# Autodesk Inventor assembly: nc_nhk8
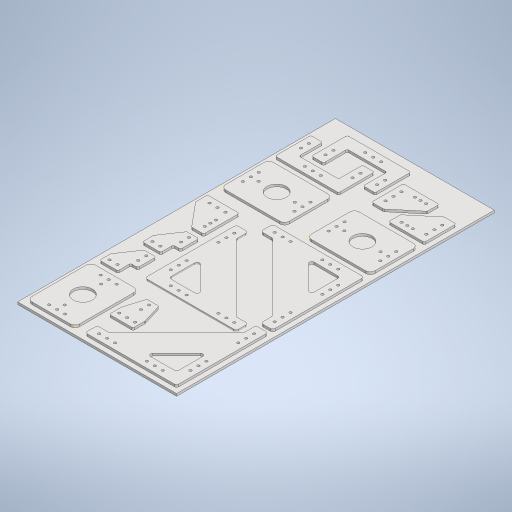
[picture p0: Inventor's stored thumbnail of the model, 512x512]
Saved by Autodesk Inventor 2023 (Build 270158000, 158)
## iProperties
Created: 2022-04-21
Part Number: nc_nhk8
Document SubType Name: Assembly
Designer: yuta
Author: yuta
## Documents named in this file (8)
- C:\Users\yuta\Documents\NHK\nc_nhk8.iam
- C:\Users\yuta\Documents\NHK\NC.port.ipt
- C:\Users\yuta\Documents\NHK\射出_エンコーダー固定.ipt
- C:\Users\yuta\Documents\NHK\射出_固定5.ipt
- C:\Users\yuta\Documents\NHK\射出_固定4.ipt
- C:\Users\yuta\Documents\NHK\射出_固定2.ipt
- C:\Users\yuta\Documents\NHK\射出_固定3.ipt
- C:\Users\yuta\Documents\NHK\射出_固定1.ipt
## Components (15 placed, 7 different names)
1. NC.port:1 — メイト:1, フラッシュ:1, フラッシュ:2, メイト:2, フラッシュ:3, フラッシュ:4, メイト:5, メイト:8, フラッシュ:5, メイト:12, メイト:14, メイト:17, フラッシュ:6, メイト:19, フラッシュ:7, メイト:21, フラッシュ:8, メイト:23, フラッシュ:9, メイト:25, メイト:28, メイト:30, フラッシュ:10
2. 射出_固定5:1 — メイト:5, メイト:6, メイト:7, メイト:10
3. 射出_固定2:1 — メイト:2, フラッシュ:3, フラッシュ:4, メイト:7, メイト:9, メイト:11
4. 射出_エンコーダー固定:1 — メイト:1, フラッシュ:1, フラッシュ:2, メイト:6, メイト:13
5. 射出_固定2:2 — メイト:8, フラッシュ:5, メイト:9, メイト:18, メイト:20
6. 射出_固定2:3 — メイト:10, メイト:11, メイト:16
7. 射出_固定4:1 — メイト:14, メイト:15, メイト:16, メイト:22
8. 射出_固定4:2 — メイト:12, メイト:13, メイト:15
9. 射出_エンコーダー固定:2 — メイト:17, フラッシュ:6, メイト:18, メイト:24
10. 射出_エンコーダー固定:3 — メイト:19, フラッシュ:7, メイト:20, メイト:31
11. 射出_固定3:1 — メイト:21, フラッシュ:8, メイト:22
12. 射出_固定3:2 — メイト:30, フラッシュ:10, メイト:31
13. 射出_固定3:3 — メイト:28, メイト:29
14. 射出_固定1:1 — メイト:25, メイト:26, メイト:27, メイト:29
15. 射出_固定1:2 — メイト:23, メイト:24, フラッシュ:9, メイト:26, メイト:27
## Relationships (39: Mate 29, Flush 10)
- メイト:1 [Mate]: NC.port:1 ↔ 射出_エンコーダー固定:1
- フラッシュ:1 [Flush] (6 mm): NC.port:1 ↔ 射出_エンコーダー固定:1
- フラッシュ:2 [Flush] (6 mm): NC.port:1 ↔ 射出_エンコーダー固定:1
- メイト:2 [Mate]: NC.port:1 ↔ 射出_固定2:1
- フラッシュ:3 [Flush] (6 mm): NC.port:1 ↔ 射出_固定2:1
- フラッシュ:4 [Flush] (6 mm): NC.port:1 ↔ 射出_固定2:1
- メイト:5 [Mate]: NC.port:1 ↔ 射出_固定5:1
- メイト:6 [Mate] (8 mm): 射出_固定5:1 ↔ 射出_エンコーダー固定:1
- メイト:7 [Mate] (10 mm): 射出_固定5:1 ↔ 射出_固定2:1
- メイト:8 [Mate]: NC.port:1 ↔ 射出_固定2:2
- フラッシュ:5 [Flush] (6 mm): NC.port:1 ↔ 射出_固定2:2
- メイト:9 [Mate] (6 mm): 射出_固定2:1 ↔ 射出_固定2:2
- メイト:10 [Mate] (23 mm): 射出_固定5:1 ↔ 射出_固定2:3
- メイト:11 [Mate] (8 mm): 射出_固定2:1 ↔ 射出_固定2:3
- メイト:12 [Mate]: NC.port:1 ↔ 射出_固定4:2
- メイト:13 [Mate] (8 mm): 射出_エンコーダー固定:1 ↔ 射出_固定4:2
- メイト:14 [Mate]: NC.port:1 ↔ 射出_固定4:1
- メイト:15 [Mate] (8 mm): 射出_固定4:1 ↔ 射出_固定4:2
- メイト:16 [Mate] (8 mm): 射出_固定2:3 ↔ 射出_固定4:1
- メイト:17 [Mate]: NC.port:1 ↔ 射出_エンコーダー固定:2
- フラッシュ:6 [Flush] (6 mm): NC.port:1 ↔ 射出_エンコーダー固定:2
- メイト:18 [Mate] (8 mm): 射出_固定2:2 ↔ 射出_エンコーダー固定:2
- メイト:19 [Mate]: NC.port:1 ↔ 射出_エンコーダー固定:3
- フラッシュ:7 [Flush] (6 mm): NC.port:1 ↔ 射出_エンコーダー固定:3
- メイト:20 [Mate] (8 mm): 射出_固定2:2 ↔ 射出_エンコーダー固定:3
- メイト:21 [Mate]: NC.port:1 ↔ 射出_固定3:1
- フラッシュ:8 [Flush] (6 mm): NC.port:1 ↔ 射出_固定3:1
- メイト:22 [Mate] (8 mm): 射出_固定4:1 ↔ 射出_固定3:1
- メイト:23 [Mate]: NC.port:1 ↔ 射出_固定1:2
- メイト:24 [Mate] (8 mm): 射出_エンコーダー固定:2 ↔ 射出_固定1:2
- フラッシュ:9 [Flush] (6 mm): NC.port:1 ↔ 射出_固定1:2
- メイト:25 [Mate]: NC.port:1 ↔ 射出_固定1:1
- メイト:26 [Mate] (8 mm): 射出_固定1:1 ↔ 射出_固定1:2
- メイト:27 [Mate] (8 mm): 射出_固定1:1 ↔ 射出_固定1:2
- メイト:28 [Mate]: NC.port:1 ↔ 射出_固定3:3
- メイト:29 [Mate] (8 mm): 射出_固定3:3 ↔ 射出_固定1:1
- メイト:30 [Mate]: NC.port:1 ↔ 射出_固定3:2
- フラッシュ:10 [Flush] (6 mm): NC.port:1 ↔ 射出_固定3:2
- メイト:31 [Mate] (8 mm): 射出_エンコーダー固定:3 ↔ 射出_固定3:2
